# Autodesk Inventor assembly: frame assembly 5
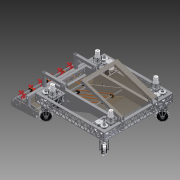
[picture p0: Inventor's stored thumbnail of the model, 180x180]
Saved by Autodesk Inventor 2012 (Build 160160000, 160)
## iProperties
Created: 2013-07-06
Part Number: frame assembly 5
Document SubType Name: Assembly
Designer: Bryce
Author: Bryce
## Documents named in this file (28)
- C:\Users\Bryce\Dropbox\Inventor Design Project Files\Independent Swerves\Inventor 2012\frame assembly 5.iam
- C:\Users\Bryce\Dropbox\Inventor Design Project Files\Independent Swerves\Inventor 2012\big U channel 3.25in.ipt
- C:\Users\Bryce\Dropbox\Inventor Design Project Files\Independent Swerves\Inventor 2012\FULL SWERVE DRIVE ASSEMBLY!  2!.iam
- C:\Users\Bryce\Dropbox\Inventor Design Project Files\Independent Swerves\Inventor 2012\frame tube 1 by 3in.ipt
- C:\Users\Bryce\Dropbox\Inventor Design Project Files\Independent Swerves\Inventor 2012\apendage bearing braket.ipt
- C:\Users\Bryce\Dropbox\Inventor Design Project Files\Independent Swerves\Inventor 2012\apendage horisantal arm.ipt
- C:\Users\Bryce\Dropbox\Inventor Design Project Files\Independent Swerves\Inventor 2012\apendage vertical arm.ipt
- C:\Users\Bryce\Dropbox\Inventor Design Project Files\Independent Swerves\Inventor 2012\apendage widening tube.ipt
- C:\Users\Bryce\Dropbox\Inventor Design Project Files\Independent Swerves\Inventor 2012\apendage motor bracket.ipt
- C:\Users\Bryce\Dropbox\Inventor Design Project Files\Independent Swerves\Inventor 2012\main intake shaft.ipt
- C:\Users\Bryce\Dropbox\Inventor Design Project Files\Independent Swerves\Inventor 2012\rubber intake star.ipt
- C:\Users\Bryce\Dropbox\Inventor Design Project Files\Independent Swerves\Inventor 2012\polycarb apendage bottom.ipt
- C:\Users\Bryce\Dropbox\Inventor Design Project Files\Independent Swerves\Imported Components\0.5'' 15 tooth flange threaded.ipt
- C:\Users\Bryce\Dropbox\Inventor Design Project Files\Inventor library\Sprockets_Belt\32-5m15-6a3.ipt
- C:\Users\Bryce\Dropbox\Inventor Design Project Files\Independent Swerves\Inventor 2012\apendage polycord shaft.ipt
- C:\Users\Bryce\Dropbox\Inventor Design Project Files\Independent Swerves\Inventor 2012\polycord pully.ipt
- C:\Users\Bryce\Dropbox\Inventor Design Project Files\Independent Swerves\Inventor 2012\apendage polycarb wedge.ipt
- C:\Users\Bryce\Dropbox\Inventor Design Project Files\Independent Swerves\Inventor 2012\uptake bearing plate.ipt
- C:\Users\Bryce\Dropbox\Inventor Design Project Files\Independent Swerves\Inventor 2012\polycarb uptake bottom.ipt
- C:\Users\Bryce\Dropbox\Inventor Design Project Files\Independent Swerves\Inventor 2012\uptake support bracket.ipt
- C:\Users\Bryce\Dropbox\Inventor Design Project Files\Independent Swerves\Inventor 2012\uptake polycord shaft.ipt
- C:\Users\Bryce\Dropbox\Inventor Design Project Files\Independent Swerves\Inventor 2012\uptake polycord.ipt
- C:\Users\Bryce\Dropbox\Inventor Design Project Files\Independent Swerves\Inventor 2012\apendage polycord.ipt
- C:\Users\Bryce\Dropbox\Inventor Design Project Files\Independent Swerves\Inventor 2012\shooter frame tube.ipt
- C:\Users\Bryce\Dropbox\Inventor Design Project Files\Independent Swerves\Inventor 2012\shooter bearing bracket.ipt
- C:\Users\Bryce\Dropbox\Inventor Design Project Files\Independent Swerves\Inventor 2012\shooter U frame.ipt
- C:\Users\Bryce\Dropbox\Inventor Design Project Files\Independent Swerves\Inventor 2012\shooter cross tube.ipt
- C:\Users\Bryce\Dropbox\Inventor Design Project Files\Independent Swerves\Inventor 2012\polycarb shooter bottom.ipt
## Components (66 placed, 27 different names)
1. big U channel 3.25in:1 — Flush:1, Mate:1, Mate:2, Mate:4, Mate:13, Mate:14, Mate:19, Mate:20, Mate:22, Mate:23, Flush:8, Mate:92, Mate:96, Mate:132
2. big U channel 3.25in:2 — Flush:2, Flush:3, Mate:3, Mate:8, Mate:10, Mate:12, Mate:16, Mate:94, Mate:97, Flush:46, Flush:47, Mate:135, Mate:136
3. big U channel 3.25in:3 — Flush:3, Mate:2, Mate:5, Mate:11, Mate:12, Mate:13, Mate:17, Mate:146
4. big U channel 3.25in:4 — Flush:1, Flush:2, Mate:1, Mate:3, Mate:9, Mate:14, Mate:15, Mate:100, Mate:131, Mate:133
5. FULL SWERVE DRIVE ASSEMBLY!  2!:1 [sub-assembly] — Mate:4, Mate:5, Mate:17, Mate:24
6. FULL SWERVE DRIVE ASSEMBLY!  2!:3 [sub-assembly] — Mate:10, Mate:11, Mate:16
7. FULL SWERVE DRIVE ASSEMBLY!  2!:4 [sub-assembly] — Mate:8, Mate:9, Mate:15
8. frame tube 1 by 3in:1 — Mate:19, Mate:20, Mate:25, Mate:27, Mate:91, Mate:95, Mate:100, Angle:2, Mate:113, Mate:138, Angle:122
9. frame tube 1 by 3in:2 — Mate:22, Mate:23, Mate:24, Mate:26, Mate:28, Mate:90, Mate:93, Angle:1, Mate:106, Mate:112, Mate:137, Mate:146
10. apendage bearing braket:1 — Mate:25, Flush:6, Mate:27, Mate:29, Mate:30, Flush:8
11. apendage bearing braket:2 — Mate:26, Flush:6, Mate:28, Mate:31, Mate:32
12. apendage horisantal arm:1 — Mate:29, Mate:30, Flush:7, Mate:34, Flush:11, Flush:12, Angle:122
13. apendage horisantal arm:2 — Mate:31, Mate:32, Flush:7, Mate:33, Flush:9, Flush:10
14. apendage vertical arm:1 — Mate:33, Flush:9, Flush:10, Flush:14, Mate:35
15. apendage vertical arm:2 — Mate:34, Flush:11, Flush:12, Flush:29
16. apendage widening tube:2 — Flush:14, Mate:35, Flush:17, Flush:18, Mate:37, Flush:29, Mate:60, Flush:30, Flush:31
17. apendage vertical arm:3 — Mate:40, Mate:60, Flush:30, Flush:31, Mate:64, Mate:65
18. apendage vertical arm:4 — Flush:17, Flush:18, Mate:37, Mate:61, Mate:62, Mate:145
19. apendage motor bracket:1 — Mate:40, Flush:28, Mate:58, Mate:59, Flush:32, Mate:64, Mate:65, Mate:66, Flush:33, Mate:89
20. main intake shaft:1 — Mate:46, Mate:47, Mate:48, Mate:49, Mate:50, Mate:51, Mate:66, Flush:33, Mate:70, Mate:74, Mate:75, Mate:76
21. rubber intake star:1 — Mate:46, Flush:23, Mate:53, Mate:67
22. rubber intake star:2 — Mate:47, Flush:23, Flush:24, Mate:53, Mate:54, Mate:83
23. rubber intake star:3 — Mate:48, Flush:24, Flush:25, Mate:54, Mate:55
24. rubber intake star:4 — Mate:49, Flush:25, Flush:26, Mate:57
25. rubber intake star:5 — Mate:50, Flush:26, Flush:27, Mate:55, Mate:56
26. rubber intake star:6 — Mate:51, Flush:27, Mate:56, Mate:57, Mate:84
27. polycarb apendage bottom:1 — Flush:28, Mate:58, Mate:59, Mate:86, Mate:88
28. apendage motor bracket:2 — Mate:61, Mate:62, Flush:32, Mate:67, Mate:68, Mate:69, Mate:71, Mate:72, Mate:73, Flush:34, Flush:35, Mate:85, Mate:87, Flush:43, Mate:145
29. 0.5'' 15 tooth flange threaded:1 — Mate:68, Mate:69
30. 32-5m15-6a3:1 — Mate:70, Mate:71
31. apendage polycord shaft:1 — Mate:72, Flush:34, Mate:77, Mate:78, Mate:79
32. apendage polycord shaft:2 — Mate:73, Flush:35, Mate:80, Mate:81, Mate:82
33. polycord pully:1 — Mate:74, Flush:38, Flush:39, Mate:85
34. polycord pully:2 — Mate:75, Flush:36, Mate:83
35. polycord pully:3 — Mate:76, Flush:40, Mate:84
36. polycord pully:4 — Mate:77, Flush:36, Flush:37, Mate:129
37. polycord pully:5 — Mate:78, Flush:38, Mate:128
38. polycord pully:6 — Mate:79, Flush:40, Flush:41, Mate:130
39. polycord pully:7 — Mate:82, Flush:37, Mate:124, Mate:125
40. polycord pully:8 — Mate:81, Flush:41, Mate:126, Mate:127
41. polycord pully:9 — Mate:80, Flush:39, Mate:122, Mate:123
42. apendage polycarb wedge:1 — Mate:86, Mate:87, Flush:42, Flush:43
43. apendage polycarb wedge:2 — Mate:88, Mate:89, Flush:42
44. uptake bearing plate:1 — Mate:90, Mate:92, Mate:93, Mate:94, Mate:98, Mate:99, Flush:44, Mate:101, Mate:102, Mate:105, Mate:107, Mate:114, Angle:120
45. uptake bearing plate:2 — Mate:91, Mate:95, Mate:96, Mate:97, Mate:103, Mate:104, Flush:45, Mate:115, Angle:121
46. polycarb uptake bottom:1 — Mate:98, Mate:99, Flush:44
47. uptake support bracket:1 — Mate:101, Mate:102, Angle:1
48. uptake support bracket:2 — Mate:103, Mate:104, Angle:2
49. uptake polycord shaft:1 — Mate:106, Mate:107, Mate:110, Mate:111
50. uptake polycord shaft:2 — Mate:105, Flush:45, Mate:108, Mate:109
51. polycord pully:10 — Mate:109, Mate:115
52. polycord pully:11 — Mate:108, Mate:114
53. polycord pully:12 — Mate:110, Mate:112, Mate:116, Mate:117
54. polycord pully:13 — Mate:111, Mate:113, Mate:118, Mate:119
55. uptake polycord:1 — Mate:116, Mate:117, Angle:120
56. uptake polycord:2 — Mate:118, Mate:119, Angle:121
57. apendage polycord:1 — Mate:126, Mate:127, Mate:130
58. apendage polycord:2 — Mate:122, Mate:123, Mate:128
59. apendage polycord:3 — Mate:124, Mate:125, Mate:129
60. FULL SWERVE DRIVE ASSEMBLY!  2!:5 [sub-assembly] — Mate:131, Mate:132, Mate:133
61. apendage bearing braket:3 — Flush:46, Mate:135, Mate:138, Mate:139, Mate:140
62. shooter bearing bracket:1 — Flush:47, Mate:136, Mate:137, Mate:141, Mate:142
63. shooter frame tube:1 — Mate:139, Mate:140, Flush:49
64. shooter U frame:1 — Mate:141, Mate:142, Flush:49, Mate:143, Flush:50, Flush:51, Mate:144, Flush:52, Flush:53
65. shooter cross tube:1 — Mate:143, Flush:50, Flush:51
66. polycarb shooter bottom:1 — Mate:144, Flush:52, Flush:53
## Relationships (177: Mate 129, Flush 43, Angle 5)
- Flush:1: big U channel 3.25in:1 ↔ big U channel 3.25in:4
- Flush:2: big U channel 3.25in:2 ↔ big U channel 3.25in:4
- Flush:3: big U channel 3.25in:2 ↔ big U channel 3.25in:3
- Mate:1: big U channel 3.25in:1 ↔ big U channel 3.25in:4
- Mate:2: big U channel 3.25in:1 ↔ big U channel 3.25in:3
- Mate:3: big U channel 3.25in:2 ↔ big U channel 3.25in:4
- Mate:4: big U channel 3.25in:1 ↔ FULL SWERVE DRIVE ASSEMBLY!  2!:1
- Mate:5: big U channel 3.25in:3 ↔ FULL SWERVE DRIVE ASSEMBLY!  2!:1
- Mate:8: big U channel 3.25in:2 ↔ FULL SWERVE DRIVE ASSEMBLY!  2!:4
- Mate:9: big U channel 3.25in:4 ↔ FULL SWERVE DRIVE ASSEMBLY!  2!:4
- Mate:10: big U channel 3.25in:2 ↔ FULL SWERVE DRIVE ASSEMBLY!  2!:3
- Mate:11: big U channel 3.25in:3 ↔ FULL SWERVE DRIVE ASSEMBLY!  2!:3
- Mate:12: big U channel 3.25in:2 ↔ big U channel 3.25in:3
- Mate:13: big U channel 3.25in:1 ↔ big U channel 3.25in:3
- Mate:14: big U channel 3.25in:1 ↔ big U channel 3.25in:4
- Mate:15: big U channel 3.25in:4 ↔ FULL SWERVE DRIVE ASSEMBLY!  2!:4
- Mate:16: big U channel 3.25in:2 ↔ FULL SWERVE DRIVE ASSEMBLY!  2!:3
- Mate:17: big U channel 3.25in:3 ↔ FULL SWERVE DRIVE ASSEMBLY!  2!:1
- Mate:19: big U channel 3.25in:1 ↔ frame tube 1 by 3in:1
- Mate:20: big U channel 3.25in:1 ↔ frame tube 1 by 3in:1
- Mate:22: big U channel 3.25in:1 ↔ frame tube 1 by 3in:2
- Mate:23: big U channel 3.25in:1 ↔ frame tube 1 by 3in:2
- Mate:24 (22.225 mm): FULL SWERVE DRIVE ASSEMBLY!  2!:1 ↔ frame tube 1 by 3in:2
- Mate:25: frame tube 1 by 3in:1 ↔ apendage bearing braket:1
- Mate:26: frame tube 1 by 3in:2 ↔ apendage bearing braket:2
- Flush:6: apendage bearing braket:1 ↔ apendage bearing braket:2
- Mate:27: frame tube 1 by 3in:1 ↔ apendage bearing braket:1
- Mate:28: frame tube 1 by 3in:2 ↔ apendage bearing braket:2
- Mate:29: apendage bearing braket:1 ↔ apendage horisantal arm:1
- Mate:30: apendage bearing braket:1 ↔ apendage horisantal arm:1
- Mate:31: apendage bearing braket:2 ↔ apendage horisantal arm:2
- Mate:32: apendage bearing braket:2 ↔ apendage horisantal arm:2
- Flush:7: apendage horisantal arm:1 ↔ apendage horisantal arm:2
- Flush:8 (76.2 mm): big U channel 3.25in:1 ↔ apendage bearing braket:1
- Mate:33: apendage horisantal arm:2 ↔ apendage vertical arm:1
- Flush:9: apendage horisantal arm:2 ↔ apendage vertical arm:1
- Flush:10: apendage horisantal arm:2 ↔ apendage vertical arm:1
- Mate:34: apendage horisantal arm:1 ↔ apendage vertical arm:2
- Flush:11: apendage horisantal arm:1 ↔ apendage vertical arm:2
- Flush:12: apendage horisantal arm:1 ↔ apendage vertical arm:2
- Flush:14: apendage vertical arm:1 ↔ apendage widening tube:2
- Mate:35: apendage vertical arm:1 ↔ apendage widening tube:2
- Flush:17: apendage widening tube:2 ↔ apendage vertical arm:4
- Flush:18: apendage widening tube:2 ↔ apendage vertical arm:4
- Mate:37: apendage widening tube:2 ↔ apendage vertical arm:4
- Mate:40: apendage vertical arm:3 ↔ apendage motor bracket:1
- Mate:46: main intake shaft:1 ↔ rubber intake star:1
- Mate:47: main intake shaft:1 ↔ rubber intake star:2
- Mate:48: main intake shaft:1 ↔ rubber intake star:3
- Mate:49: main intake shaft:1 ↔ rubber intake star:4
- Mate:50: main intake shaft:1 ↔ rubber intake star:5
- Mate:51: main intake shaft:1 ↔ rubber intake star:6
- Flush:23: rubber intake star:1 ↔ rubber intake star:2
- Flush:24: rubber intake star:2 ↔ rubber intake star:3
- Flush:25: rubber intake star:3 ↔ rubber intake star:4
- Flush:26: rubber intake star:4 ↔ rubber intake star:5
- Flush:27: rubber intake star:5 ↔ rubber intake star:6
- Mate:53 (86.868 mm): rubber intake star:1 ↔ rubber intake star:2
- Mate:54 (86.868 mm): rubber intake star:2 ↔ rubber intake star:3
- Mate:55 (86.868 mm): rubber intake star:3 ↔ rubber intake star:5
- Mate:56 (86.868 mm): rubber intake star:5 ↔ rubber intake star:6
- Mate:57 (86.868 mm): rubber intake star:4 ↔ rubber intake star:6
- Flush:28: apendage motor bracket:1 ↔ polycarb apendage bottom:1
- Mate:58: apendage motor bracket:1 ↔ polycarb apendage bottom:1
- Mate:59: apendage motor bracket:1 ↔ polycarb apendage bottom:1
- Flush:29 (-165.1 mm): apendage vertical arm:2 ↔ apendage widening tube:2
- Mate:60: apendage widening tube:2 ↔ apendage vertical arm:3
- Flush:30: apendage widening tube:2 ↔ apendage vertical arm:3
- Flush:31: apendage widening tube:2 ↔ apendage vertical arm:3
- Mate:61: apendage vertical arm:4 ↔ apendage motor bracket:2
- Mate:62: apendage vertical arm:4 ↔ apendage motor bracket:2
- Flush:32: apendage motor bracket:1 ↔ apendage motor bracket:2
- Mate:64: apendage vertical arm:3 ↔ apendage motor bracket:1
- Mate:65 (-12.7 mm): apendage vertical arm:3 ↔ apendage motor bracket:1
- Mate:66: apendage motor bracket:1 ↔ main intake shaft:1
- Flush:33 (-3.175 mm): apendage motor bracket:1 ↔ main intake shaft:1
- Mate:67 (86.868 mm): rubber intake star:1 ↔ apendage motor bracket:2
- Mate:68: apendage motor bracket:2 ↔ 0.5'' 15 tooth flange threaded:1
- Mate:69: apendage motor bracket:2 ↔ 0.5'' 15 tooth flange threaded:1
- Mate:70: main intake shaft:1 ↔ 32-5m15-6a3:1
- Mate:71: apendage motor bracket:2 ↔ 32-5m15-6a3:1
- Mate:72: apendage motor bracket:2 ↔ apendage polycord shaft:1
- Mate:73: apendage motor bracket:2 ↔ apendage polycord shaft:2
- Flush:34: apendage motor bracket:2 ↔ apendage polycord shaft:1
- Flush:35: apendage motor bracket:2 ↔ apendage polycord shaft:2
- Mate:74: main intake shaft:1 ↔ polycord pully:1
- Mate:75: main intake shaft:1 ↔ polycord pully:2
- Mate:76: main intake shaft:1 ↔ polycord pully:3
- Mate:77: apendage polycord shaft:1 ↔ polycord pully:4
- Mate:78: apendage polycord shaft:1 ↔ polycord pully:5
- Mate:79: apendage polycord shaft:1 ↔ polycord pully:6
- Mate:80: apendage polycord shaft:2 ↔ polycord pully:9
- Mate:81: apendage polycord shaft:2 ↔ polycord pully:8
- Mate:82: apendage polycord shaft:2 ↔ polycord pully:7
- Flush:36: polycord pully:2 ↔ polycord pully:4
- Flush:37: polycord pully:4 ↔ polycord pully:7
- Flush:38: polycord pully:1 ↔ polycord pully:5
- Flush:39: polycord pully:1 ↔ polycord pully:9
- Flush:40: polycord pully:3 ↔ polycord pully:6
- Flush:41: polycord pully:6 ↔ polycord pully:8
- Mate:83: rubber intake star:2 ↔ polycord pully:2
- Mate:84: rubber intake star:6 ↔ polycord pully:3
- Mate:85 (307.975 mm): apendage motor bracket:2 ↔ polycord pully:1
- Mate:86: polycarb apendage bottom:1 ↔ apendage polycarb wedge:1
- Mate:87: apendage motor bracket:2 ↔ apendage polycarb wedge:1
- Mate:88: polycarb apendage bottom:1 ↔ apendage polycarb wedge:2
- Mate:89: apendage motor bracket:1 ↔ apendage polycarb wedge:2
- Flush:42: apendage polycarb wedge:1 ↔ apendage polycarb wedge:2
- Flush:43 (31.75 mm): apendage motor bracket:2 ↔ apendage polycarb wedge:1
- Mate:90: frame tube 1 by 3in:2 ↔ uptake bearing plate:1
- Mate:91: frame tube 1 by 3in:1 ↔ uptake bearing plate:2
- Mate:92: big U channel 3.25in:1 ↔ uptake bearing plate:1
- Mate:93: frame tube 1 by 3in:2 ↔ uptake bearing plate:1
- Mate:94 (304.8 mm): big U channel 3.25in:2 ↔ uptake bearing plate:1
- Mate:95: frame tube 1 by 3in:1 ↔ uptake bearing plate:2
- Mate:96: big U channel 3.25in:1 ↔ uptake bearing plate:2
- Mate:97 (304.8 mm): big U channel 3.25in:2 ↔ uptake bearing plate:2
- Mate:98: uptake bearing plate:1 ↔ polycarb uptake bottom:1
- Mate:99: uptake bearing plate:1 ↔ polycarb uptake bottom:1
- Flush:44: uptake bearing plate:1 ↔ polycarb uptake bottom:1
- Mate:100 (177.8 mm): big U channel 3.25in:4 ↔ frame tube 1 by 3in:1
- Mate:101: uptake bearing plate:1 ↔ uptake support bracket:1
- Mate:102: uptake bearing plate:1 ↔ uptake support bracket:1
- Angle:1 (180 deg): frame tube 1 by 3in:2 ↔ uptake support bracket:1
- Mate:103: uptake bearing plate:2 ↔ uptake support bracket:2
- Mate:104: uptake bearing plate:2 ↔ uptake support bracket:2
- Angle:2 (180 deg): frame tube 1 by 3in:1 ↔ uptake support bracket:2
- Mate:105: uptake bearing plate:1 ↔ uptake polycord shaft:2
- Flush:45: uptake bearing plate:2 ↔ uptake polycord shaft:2
- Mate:106: frame tube 1 by 3in:2 ↔ uptake polycord shaft:1
- Mate:107: uptake bearing plate:1 ↔ uptake polycord shaft:1
- Mate:108: uptake polycord shaft:2 ↔ polycord pully:11
- Mate:109: uptake polycord shaft:2 ↔ polycord pully:10
- Mate:110: uptake polycord shaft:1 ↔ polycord pully:12
- Mate:111: uptake polycord shaft:1 ↔ polycord pully:13
- Mate:112 (92.964 mm): frame tube 1 by 3in:2 ↔ polycord pully:12
- Mate:113 (92.964 mm): frame tube 1 by 3in:1 ↔ polycord pully:13
- Mate:114 (92.964 mm): uptake bearing plate:1 ↔ polycord pully:11
- Mate:115 (92.964 mm): uptake bearing plate:2 ↔ polycord pully:10
- Mate:116: polycord pully:12 ↔ uptake polycord:1
- Mate:117 (-6.35 mm): polycord pully:12 ↔ uptake polycord:1
- Mate:118: polycord pully:13 ↔ uptake polycord:2
- Mate:119 (-6.35 mm): polycord pully:13 ↔ uptake polycord:2
- Angle:120 (-90 deg): uptake bearing plate:1 ↔ uptake polycord:1
- Angle:121 (90 deg): uptake bearing plate:2 ↔ uptake polycord:2
- Mate:122: polycord pully:9 ↔ apendage polycord:2
- Mate:123 (-6.35 mm): polycord pully:9 ↔ apendage polycord:2
- Mate:124: polycord pully:7 ↔ apendage polycord:3
- Mate:125 (-6.35 mm): polycord pully:7 ↔ apendage polycord:3
- Mate:126: polycord pully:8 ↔ apendage polycord:1
- Mate:127 (-6.35 mm): polycord pully:8 ↔ apendage polycord:1
- Mate:128: polycord pully:5 ↔ apendage polycord:2
- Mate:129: polycord pully:4 ↔ apendage polycord:3
- Mate:130: polycord pully:6 ↔ apendage polycord:1
- Mate:131: big U channel 3.25in:4 ↔ FULL SWERVE DRIVE ASSEMBLY!  2!:5
- Mate:132: big U channel 3.25in:1 ↔ FULL SWERVE DRIVE ASSEMBLY!  2!:5
- Mate:133: big U channel 3.25in:4 ↔ FULL SWERVE DRIVE ASSEMBLY!  2!:5
- Flush:46: big U channel 3.25in:2 ↔ apendage bearing braket:3
- Flush:47: big U channel 3.25in:2 ↔ shooter bearing bracket:1
- Mate:135: big U channel 3.25in:2 ↔ apendage bearing braket:3
- Mate:136: big U channel 3.25in:2 ↔ shooter bearing bracket:1
- Mate:137: frame tube 1 by 3in:2 ↔ shooter bearing bracket:1
- Mate:138: frame tube 1 by 3in:1 ↔ apendage bearing braket:3
- Mate:139: apendage bearing braket:3 ↔ shooter frame tube:1
- Mate:140: apendage bearing braket:3 ↔ shooter frame tube:1
- Mate:141: shooter bearing bracket:1 ↔ shooter U frame:1
- Mate:142: shooter bearing bracket:1 ↔ shooter U frame:1
- Flush:49: shooter frame tube:1 ↔ shooter U frame:1
- Mate:143: shooter U frame:1 ↔ shooter cross tube:1
- Flush:50: shooter U frame:1 ↔ shooter cross tube:1
- Flush:51: shooter U frame:1 ↔ shooter cross tube:1
- Mate:144: shooter U frame:1 ↔ polycarb shooter bottom:1
- Flush:52: shooter U frame:1 ↔ polycarb shooter bottom:1
- Flush:53: shooter U frame:1 ↔ polycarb shooter bottom:1
- Angle:122 (0 deg): frame tube 1 by 3in:1 ↔ apendage horisantal arm:1
- Mate:145 (-12.7 mm): apendage vertical arm:4 ↔ apendage motor bracket:2
- Mate:146 (177.8 mm): big U channel 3.25in:3 ↔ frame tube 1 by 3in:2
